# Autodesk Inventor assembly: Assembly_Cube_SEEED_Xiao_Sense_Camera_v3
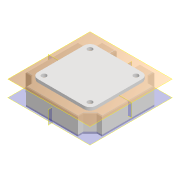
[picture p0: Inventor's stored thumbnail of the model, 180x180]
Saved by Autodesk Inventor 2022 (Build 260153000, 153)
## iProperties
Created: 2023-04-26
Part Number: Assembly_Cube_SEEED_Xiao_Sense_Camera_v3
Document SubType Name: Assembly
Designer: diederichbenedict
Author: diederichbenedict
## Documents named in this file (4)
- C:\Users\diederichbenedict\Dropbox\Dokumente\Promotion\PROJECTS\openUC2-CAD\INVENTOR\Assembly_Cube_SEEED_Xiao_Sense_Camera_v3.iam
- C:\Users\diederichbenedict\Dropbox\Dokumente\Promotion\PROJECTS\openUC2-CAD\INVENTOR\00_Seeeduino Xiao.ipt
- C:\Users\diederichbenedict\Dropbox\Dokumente\Promotion\PROJECTS\openUC2-CAD\INVENTOR\20_Cube_Insert_SEEED_Xiao_Sense_Camera.ipt
- C:\Users\diederichbenedict\Dropbox\Dokumente\Promotion\PROJECTS\openUC2-CAD\INVENTOR\20_Cube_Insert_SEEED_Xiao_Sense_Camera_backplate.ipt
## Components (3 placed, 3 different names)
1. 00_Seeeduino Xiao:1 — Passend:1, Winkel:1, Fluchtend:3
2. 20_Cube_Insert_SEEED_Xiao_Sense_Camera:1 — Fluchtend:1, Passend:2, Fluchtend:2, Winkel:1, Fluchtend:3, Fluchtend:4, Fluchtend:5, Fluchtend:6
3. 20_Cube_Insert_SEEED_Xiao_Sense_Camera_backplate:1 — Fluchtend:4, Fluchtend:5, Fluchtend:6
## Relationships (9: Flush 6, Mate 2, Angle 1)
- Passend:1 [Mate]: 00_Seeeduino Xiao:1
- Fluchtend:1 [Flush]: 20_Cube_Insert_SEEED_Xiao_Sense_Camera:1
- Passend:2 [Mate]: 20_Cube_Insert_SEEED_Xiao_Sense_Camera:1
- Fluchtend:2 [Flush]: 20_Cube_Insert_SEEED_Xiao_Sense_Camera:1
- Winkel:1 [Angle] (180 deg): 00_Seeeduino Xiao:1 ↔ 20_Cube_Insert_SEEED_Xiao_Sense_Camera:1
- Fluchtend:3 [Flush] (5 mm): 00_Seeeduino Xiao:1 ↔ 20_Cube_Insert_SEEED_Xiao_Sense_Camera:1
- Fluchtend:4 [Flush]: 20_Cube_Insert_SEEED_Xiao_Sense_Camera:1 ↔ 20_Cube_Insert_SEEED_Xiao_Sense_Camera_backplate:1
- Fluchtend:5 [Flush]: 20_Cube_Insert_SEEED_Xiao_Sense_Camera:1 ↔ 20_Cube_Insert_SEEED_Xiao_Sense_Camera_backplate:1
- Fluchtend:6 [Flush]: 20_Cube_Insert_SEEED_Xiao_Sense_Camera:1 ↔ 20_Cube_Insert_SEEED_Xiao_Sense_Camera_backplate:1
